# Autodesk Inventor assembly: Ensamblaje2
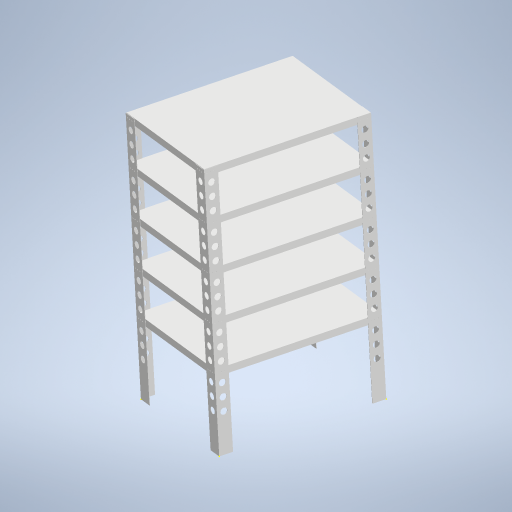
[picture p0: Inventor's stored thumbnail of the model, 512x512]
Saved by Autodesk Inventor 2024 (Build 280153000, 153)
## iProperties
Created: 2023-10-22
Part Number: Ensamblaje2
Document SubType Name: Assembly
Designer: jhonc
Author: jhonc
## Documents named in this file (3)
- C:\Users\jhonc\OneDrive\Escritorio\3 apm\estanteria\Ensamblaje2.iam
- C:\Users\jhonc\OneDrive\Escritorio\3 apm\estanteria\patas.ipt
- C:\Users\jhonc\OneDrive\Escritorio\3 apm\estanteria\secciones.ipt
## Components (9 placed, 2 different names)
1. patas:1 — Coincidencia:11, Coincidencia:12, Nivelación:1, Coincidencia:13, Coincidencia:14, Coincidencia:15, Coincidencia:16
2. secciones:1 — Coincidencia:1, Coincidencia:2, Coincidencia:4, Coincidencia:5, Coincidencia:6, Coincidencia:7, Coincidencia:8, Coincidencia:9, Coincidencia:10, Coincidencia:11, Coincidencia:12, Nivelación:1
3. patas:2 — Coincidencia:1, Coincidencia:9, Coincidencia:10, Coincidencia:17, Coincidencia:18, Coincidencia:19, Coincidencia:20
4. patas:3 — Coincidencia:4, Coincidencia:5, Coincidencia:6, Coincidencia:21, Coincidencia:22, Coincidencia:23, Coincidencia:24
5. patas:4 — Coincidencia:2, Coincidencia:7, Coincidencia:8
6. secciones:3 — Coincidencia:13, Coincidencia:20, Coincidencia:21
7. secciones:4 — Coincidencia:16, Coincidencia:17, Coincidencia:24
8. secciones:5 — Coincidencia:14, Coincidencia:19, Coincidencia:22
9. secciones:6 — Coincidencia:15, Coincidencia:18, Coincidencia:23
## Relationships (24: Mate 23, Flush 1)
- Coincidencia:1 [Mate]: secciones:1 ↔ patas:2
- Coincidencia:2 [Mate]: secciones:1 ↔ patas:4
- Coincidencia:4 [Mate]: secciones:1 ↔ patas:3
- Coincidencia:5 [Mate]: secciones:1 ↔ patas:3
- Coincidencia:6 [Mate]: secciones:1 ↔ patas:3
- Coincidencia:7 [Mate]: secciones:1 ↔ patas:4
- Coincidencia:8 [Mate]: secciones:1 ↔ patas:4
- Coincidencia:9 [Mate]: secciones:1 ↔ patas:2
- Coincidencia:10 [Mate]: secciones:1 ↔ patas:2
- Coincidencia:11 [Mate]: patas:1 ↔ secciones:1
- Coincidencia:12 [Mate]: patas:1 ↔ secciones:1
- Nivelación:1 [Flush]: patas:1 ↔ secciones:1
- Coincidencia:13 [Mate]: patas:1 ↔ secciones:3
- Coincidencia:14 [Mate]: patas:1 ↔ secciones:5
- Coincidencia:15 [Mate]: patas:1 ↔ secciones:6
- Coincidencia:16 [Mate]: patas:1 ↔ secciones:4
- Coincidencia:17 [Mate]: patas:2 ↔ secciones:4
- Coincidencia:18 [Mate]: patas:2 ↔ secciones:6
- Coincidencia:19 [Mate]: patas:2 ↔ secciones:5
- Coincidencia:20 [Mate]: patas:2 ↔ secciones:3
- Coincidencia:21 [Mate]: patas:3 ↔ secciones:3
- Coincidencia:22 [Mate]: patas:3 ↔ secciones:5
- Coincidencia:23 [Mate]: patas:3 ↔ secciones:6
- Coincidencia:24 [Mate]: patas:3 ↔ secciones:4
